# Autodesk Inventor assembly: 射出_軸
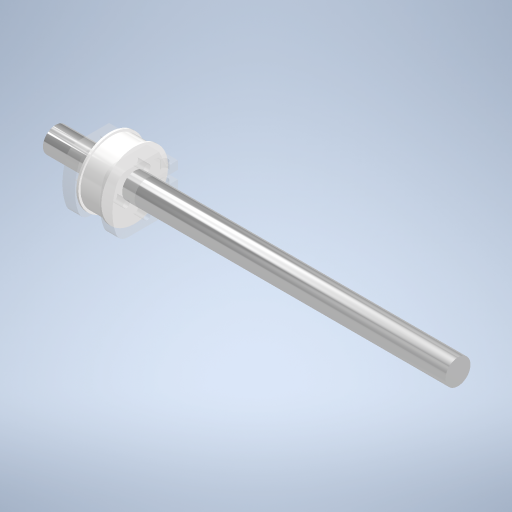
[picture p0: Inventor's stored thumbnail of the model, 512x512]
Saved by Autodesk Inventor 2023 (Build 270158000, 158)
## iProperties
Created: 2022-04-24
Part Number: 射出_軸
Document SubType Name: Assembly
Designer: yuta
Author: yuta
## Documents named in this file (4)
- C:\Users\yuta\Documents\NHK\射出_軸.iam
- C:\Users\yuta\Documents\NHK\type2.ipt
- C:\Users\yuta\Documents\NHK\射出_腕固定.ipt
- C:\Users\yuta\Documents\NHK\射出_軸.ipt
## Components (4 placed, 3 different names)
1. type2:1 — メイト:1, メイト:2, メイト:3, メイト:4, メイト:5
2. 射出_腕固定:1 — メイト:3, メイト:4, フラッシュ:1
3. 射出_腕固定:2 — メイト:1, メイト:2
4. 射出_軸:1 — メイト:5, フラッシュ:1
## Relationships (6: Mate 5, Flush 1)
- メイト:1 [Mate]: type2:1 ↔ 射出_腕固定:2
- メイト:2 [Mate]: type2:1 ↔ 射出_腕固定:2
- メイト:3 [Mate]: type2:1 ↔ 射出_腕固定:1
- メイト:4 [Mate]: type2:1 ↔ 射出_腕固定:1
- メイト:5 [Mate]: type2:1 ↔ 射出_軸:1
- フラッシュ:1 [Flush] (-20 mm): 射出_腕固定:1 ↔ 射出_軸:1
